# Autodesk Inventor assembly: 南京理工大学AllianceV3全向轮组装配
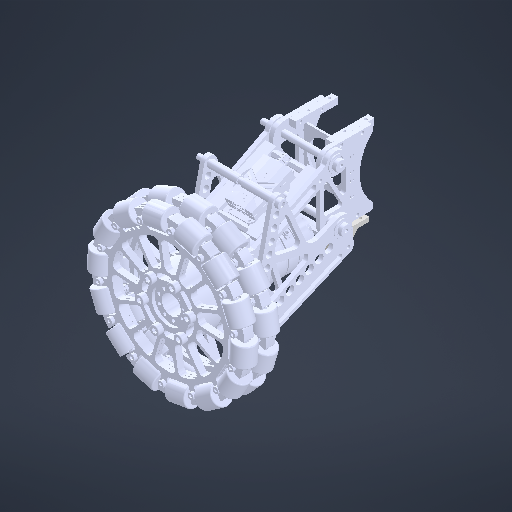
[picture p0: Inventor's stored thumbnail of the model, 512x512]
Saved by Autodesk Inventor 2025 (Build 290162000, 162)
## iProperties
Created: 2025-07-14
Part Number: 南京理工大学AllianceV3全向轮组装配
Description: STEP AP214
Document SubType Name: Assembly
Designer: XH
Sending System: SolidWorks 2024
Preprocessor: SwSTEP 2.0
Title: ÄÏ¾©Àí¹¤´óÑ§AllianceV3È«ÏòÂÖ×é×°Åä.STEP
Revision Number: ä»
## Documents named in this file (32)
- D:\gitdesktop\-\底盘\悬挂‘\南京理工大学AllianceV3全向轮组装配(1)\南京理工大学AllianceV3全向轮组装配(1).iam
- D:\gitdesktop\-\底盘\悬挂‘\南京理工大学AllianceV3全向轮组装配(1)\南京理工大学AllianceV3底盘电机座.ipt
- D:\gitdesktop\-\底盘\悬挂‘\南京理工大学AllianceV3全向轮组装配(1)\南京理工大学Alliance配件-电机3508_无线版.ipt
- D:\gitdesktop\-\底盘\悬挂‘\南京理工大学AllianceV3全向轮组装配(1)\南京理工大学Alliance垫片6x10x1.ipt
- D:\gitdesktop\-\底盘\悬挂‘\南京理工大学AllianceV3全向轮组装配(1)\南京理工大学Alliance轴承法兰6x13x5_57155K588.ipt
- D:\gitdesktop\-\底盘\悬挂‘\南京理工大学AllianceV3全向轮组装配(1)\南京理工大学AllianceV3摇臂上.ipt
- D:\gitdesktop\-\底盘\悬挂‘\南京理工大学AllianceV3全向轮组装配(1)\南京理工大学Alliance推力轴承10-26-11.ipt
- D:\gitdesktop\-\底盘\悬挂‘\南京理工大学AllianceV3全向轮组装配(1)\南京理工大学Alliance垫片10x25x2.ipt
- D:\gitdesktop\-\底盘\悬挂‘\南京理工大学AllianceV3全向轮组装配(1)\南京理工大学Alliance联轴器2.ipt
- D:\gitdesktop\-\底盘\悬挂‘\南京理工大学AllianceV3全向轮组装配(1)\南京理工大学Alliance轴套6x10x6.ipt
- D:\gitdesktop\-\底盘\悬挂‘\南京理工大学AllianceV3全向轮组装配(1)\南京理工大学Alliance不锈钢柱M3x50.ipt
- D:\gitdesktop\-\底盘\悬挂‘\南京理工大学AllianceV3全向轮组装配(1)\南京理工大学AllianceV3电调安装板.ipt
- D:\gitdesktop\-\底盘\悬挂‘\南京理工大学AllianceV3全向轮组装配(1)\南京理工大学Alliance配件-电调C620_无线版.ipt
- D:\gitdesktop\-\底盘\悬挂‘\南京理工大学AllianceV3全向轮组装配(1)\南京理工大学AllianceV3摇臂下.ipt
- D:\gitdesktop\-\底盘\悬挂‘\南京理工大学AllianceV3全向轮组装配(1)\南京理工大学AllianceV3摇臂固定板.ipt
- D:\gitdesktop\-\底盘\悬挂‘\南京理工大学AllianceV3全向轮组装配(1)\南京理工大学AllianceM5螺栓_M5-75.ipt
- D:\gitdesktop\-\底盘\悬挂‘\南京理工大学AllianceV3全向轮组装配(1)\南京理工大学Alliance尼龙隔离柱7x5x20.ipt
- D:\gitdesktop\-\底盘\悬挂‘\南京理工大学AllianceV3全向轮组装配(1)\南京理工大学Alliance尼龙隔离柱7x5x8.ipt
- D:\gitdesktop\-\底盘\悬挂‘\南京理工大学AllianceV3全向轮组装配(1)\南京理工大学Alliance塞打螺栓D6xM5x60.ipt
- D:\gitdesktop\-\底盘\悬挂‘\南京理工大学AllianceV3全向轮组装配(1)\南京理工大学Alliance塞打螺栓D6xM5x70.ipt
- D:\gitdesktop\-\底盘\悬挂‘\南京理工大学AllianceV3全向轮组装配(1)\南京理工大学Alliance转接件-4孔.ipt
- D:\gitdesktop\-\底盘\悬挂‘\南京理工大学AllianceV3全向轮组装配(1)\南京理工大学AllianceV3轮组-下摇臂中间铝块.ipt
- D:\gitdesktop\-\底盘\悬挂‘\南京理工大学AllianceV3全向轮组装配(1)\南京理工大学AllianceV3摇臂固定板中插板.ipt
- D:\gitdesktop\-\底盘\悬挂‘\南京理工大学AllianceV3全向轮组装配(1)\南京理工大学AllianceV3轮组卡弹丸垫块.ipt
- D:\gitdesktop\-\底盘\悬挂‘\南京理工大学AllianceV3全向轮组装配(1)\南京理工大学Alliance不锈钢管6x3x60.ipt
- D:\gitdesktop\-\底盘\悬挂‘\南京理工大学AllianceV3全向轮组装配(1)\南京理工大学Alliance航发全向轮装配V2.iam
- D:\gitdesktop\-\底盘\悬挂‘\南京理工大学AllianceV3全向轮组装配(1)\南京理工大学Alliance压紧盖.ipt
- D:\gitdesktop\-\底盘\悬挂‘\南京理工大学AllianceV3全向轮组装配(1)\hexagon socket head cap screws gb_GB_FASTENER_SCREWS_HSHCS M5X40-N.ipt
- D:\gitdesktop\-\底盘\悬挂‘\南京理工大学AllianceV3全向轮组装配(1)\hexagon socket head cap screws gb_GB_FASTENER_SCREWS_HSHCS M5X10-N.ipt
- D:\gitdesktop\-\底盘\悬挂‘\南京理工大学AllianceV3全向轮组装配(1)\hexagon socket head cap screws gb_GB_FASTENER_SCREWS_HSHCS M5X35-N.ipt
- D:\gitdesktop\-\底盘\悬挂链.ipt
- D:\gitdesktop\-\底盘\悬挂链_MIR.ipt
## Components (62 placed, 62 different names)
1. 南京理工大学AllianceV3底盘电机座_1
2. 南京理工大学Alliance配件-电机3508_无线版_2
3. 南京理工大学Alliance垫片6x10x1_3
4. 南京理工大学Alliance轴承法兰6x13x5_57155K588_4
5. 南京理工大学AllianceV3摇臂上_5
6. 南京理工大学Alliance推力轴承10-26-11_6
7. 南京理工大学Alliance垫片10x25x2_7
8. 南京理工大学Alliance联轴器2_8
9. 南京理工大学Alliance轴承法兰6x13x5_57155K588_9
10. 南京理工大学Alliance轴套6x10x6_10
11. 南京理工大学Alliance不锈钢柱M3x50_11
12. 南京理工大学Alliance不锈钢柱M3x50_12
13. 南京理工大学AllianceV3电调安装板_13
14. 南京理工大学Alliance配件-电调C620_无线版_14
15. 南京理工大学Alliance垫片6x10x1_15
16. 南京理工大学Alliance轴承法兰6x13x5_57155K588_16
17. 南京理工大学AllianceV3摇臂下_17
18. 南京理工大学Alliance轴承法兰6x13x5_57155K588_18
19. 南京理工大学Alliance轴套6x10x6_19
20. 南京理工大学AllianceV3摇臂固定板_20
21. 南京理工大学AllianceM5螺栓_M5-75_21
22. 南京理工大学Alliance尼龙隔离柱7x5x20_22
23. 南京理工大学Alliance尼龙隔离柱7x5x8_23
24. 南京理工大学AllianceV3摇臂上_24
25. 南京理工大学Alliance轴承法兰6x13x5_57155K588_25
26. 南京理工大学Alliance轴承法兰6x13x5_57155K588_26
27. 南京理工大学Alliance轴承法兰6x13x5_57155K588_27
28. 南京理工大学Alliance轴承法兰6x13x5_57155K588_28
29. 南京理工大学AllianceV3摇臂下_29
30. 南京理工大学Alliance轴套6x10x6_30
31. 南京理工大学Alliance垫片6x10x1_31
32. 南京理工大学AllianceV3摇臂固定板_32
33. 南京理工大学Alliance轴套6x10x6_33
34. 南京理工大学Alliance垫片6x10x1_34
35. 南京理工大学Alliance尼龙隔离柱7x5x20_35
36. 南京理工大学Alliance尼龙隔离柱7x5x8_36
37. 南京理工大学Alliance塞打螺栓D6xM5x60_37
38. 南京理工大学Alliance塞打螺栓D6xM5x70_38
39. 南京理工大学Alliance塞打螺栓D6xM5x60_39
40. 南京理工大学Alliance塞打螺栓D6xM5x70_40
41. 南京理工大学Alliance转接件-4孔_41 — 配合:1
42. 南京理工大学Alliance转接件-4孔_42
43. 南京理工大学Alliance转接件-4孔_43
44. 南京理工大学Alliance转接件-4孔_44
45. 南京理工大学AllianceV3轮组-下摇臂中间铝块_45
46. 南京理工大学AllianceV3摇臂固定板中插板_46
47. 南京理工大学AllianceV3轮组卡弹丸垫块_47
48. 南京理工大学Alliance不锈钢管6x3x60_48
49. 南京理工大学Alliance不锈钢管6x3x60_49
50. 南京理工大学Alliance航发全向轮装配V2_50 [sub-assembly]
51. 南京理工大学Alliance压紧盖_51
52. hexagon socket head cap screws gb_GB_FASTENER_SCREWS_HSHCS M5X40-N_52
53. hexagon socket head cap screws gb_GB_FASTENER_SCREWS_HSHCS M5X40-N_53
54. hexagon socket head cap screws gb_GB_FASTENER_SCREWS_HSHCS M5X40-N_54
55. hexagon socket head cap screws gb_GB_FASTENER_SCREWS_HSHCS M5X40-N_55
56. hexagon socket head cap screws gb_GB_FASTENER_SCREWS_HSHCS M5X40-N_56
57. hexagon socket head cap screws gb_GB_FASTENER_SCREWS_HSHCS M5X40-N_57
58. hexagon socket head cap screws gb_GB_FASTENER_SCREWS_HSHCS M5X10-N_58
59. hexagon socket head cap screws gb_GB_FASTENER_SCREWS_HSHCS M5X35-N_59
60. hexagon socket head cap screws gb_GB_FASTENER_SCREWS_HSHCS M5X35-N_60
61. 悬挂链:1 — 配合:1
62. 悬挂链_MIR:1
## Relationships (1: Mate 1)
- 配合:1 [Mate] (8 mm): 南京理工大学Alliance转接件-4孔_41 ↔ 悬挂链:1
